# Autodesk Inventor assembly: Ensamblajemotocorta
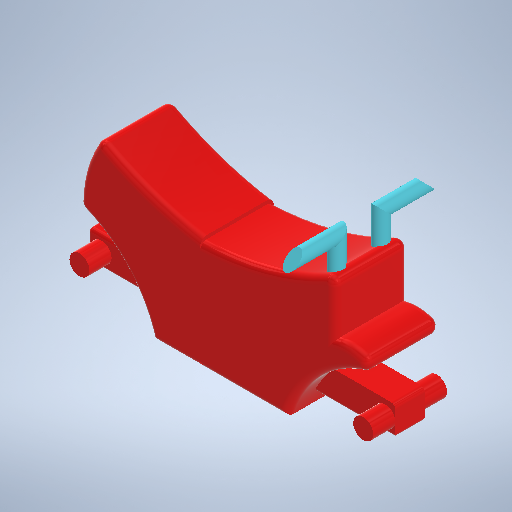
[picture p0: Inventor's stored thumbnail of the model, 512x512]
Saved by Autodesk Inventor 2025.2 (Build 292293000, 293)
## iProperties
Created: 2024-11-29
Part Number: Ensamblajemotocorta
Document SubType Name: Assembly
Designer: usuario
Author: usuario
## Documents named in this file (3)
- C:\Users\usuario\Desktop\APM\ModeladosAPM\Ensamblajemotocorta.iam
- C:\Users\usuario\Desktop\APM\ModeladosAPM\Moto - copia - copia.ipt
- C:\Users\usuario\Desktop\APM\ModeladosAPM\Moto - copia.ipt
## Components (2 placed, 2 different names)
1. Moto - copia - copia:1 — Coincidencia:1, Nivelación:1, Nivelación:2
2. Moto - copia:1 — Coincidencia:1, Nivelación:1, Nivelación:2
## Relationships (3: Flush 2, Mate 1)
- Coincidencia:1 [Mate]: Moto - copia - copia:1 ↔ Moto - copia:1
- Nivelación:1 [Flush]: Moto - copia - copia:1 ↔ Moto - copia:1
- Nivelación:2 [Flush]: Moto - copia - copia:1 ↔ Moto - copia:1
